# Autodesk Inventor assembly: Termocupla
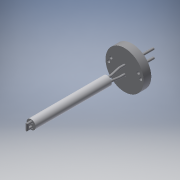
[picture p0: Inventor's stored thumbnail of the model, 180x180]
Saved by Autodesk Inventor 2017 (Build 210142000, 142)
## iProperties
Created: 2021-07-26
Part Number: Termocupla
Document SubType Name: Assembly
Designer: USUARIO
Author: USUARIO
## Documents named in this file (4)
- D:\Laboratorio\Mufla\2021\Mufla 3L Psoc Artilab #0045886XX OP2021128\Modelo\Termocupla\Termocupla.iam
- D:\Laboratorio\Mufla\2021\Mufla 3L Psoc Artilab #0045886XX OP2021128\Modelo\Termocupla\Buje.ipt
- D:\Laboratorio\Mufla\2021\Mufla 3L Psoc Artilab #0045886XX OP2021128\Modelo\Termocupla\Alambre.ipt
- D:\Laboratorio\Mufla\2021\Mufla 3L Psoc Artilab #0045886XX OP2021128\Modelo\Termocupla\cABEZOTE.ipt
## Components (3 placed, 3 different names)
1. Buje:1 — Mate:2, Mate:3, Mate:4
2. Alambre:1 — Mate:2, Mate:3, Mate:4, Mate:5
3. cABEZOTE:1 — Mate:5
## Relationships (4: Mate 4)
- Mate:2 (60 mm): Buje:1 ↔ Alambre:1
- Mate:3: Buje:1 ↔ Alambre:1
- Mate:4: Buje:1 ↔ Alambre:1
- Mate:5: Alambre:1 ↔ cABEZOTE:1
